# Autodesk Inventor assembly: test
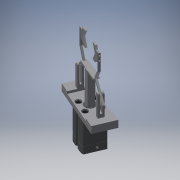
[picture p0: Inventor's stored thumbnail of the model, 180x180]
Saved by Autodesk Inventor 2017 (Build 210142000, 142)
## iProperties
Created: 2018-05-29
Part Number: test
Document SubType Name: Assembly
Designer: Pies
Author: Pies
## Documents named in this file (8)
- C:\Users\Pies\Desktop\Rzeczy\AGH\Semestr 2\ZIPK\Chwytak\Moj_Chwd_Pytak\Inventorowe chwytaki\test.iam
- C:\Users\Pies\Desktop\Rzeczy\AGH\Semestr 2\ZIPK\Chwytak\Moj_Chwd_Pytak\Inventorowe chwytaki\Ciągaczka.ipt
- C:\Users\Pies\Desktop\Rzeczy\AGH\Semestr 2\ZIPK\Chwytak\Moj_Chwd_Pytak\Inventorowe chwytaki\PIN.ipt
- C:\Users\Pies\Desktop\Rzeczy\AGH\Semestr 2\ZIPK\Chwytak\Moj_Chwd_Pytak\Inventorowe chwytaki\Ramię z łapką.iam
- C:\Users\Pies\Desktop\Rzeczy\AGH\Semestr 2\ZIPK\Chwytak\Moj_Chwd_Pytak\Inventorowe chwytaki\Podstawka.ipt
- C:\Users\Pies\Desktop\Rzeczy\AGH\Semestr 2\ZIPK\Chwytak\Moj_Chwd_Pytak\Inventorowe chwytaki\MOJ KOLNIERZ.ipt
- C:\Users\Pies\Desktop\Rzeczy\AGH\Semestr 2\ZIPK\Chwytak\Moj_Chwd_Pytak\Inventorowe chwytaki\Silownik\536236 ADN-20-15-A-P-A---(asm_0).iam
- C:\Users\Pies\Desktop\Rzeczy\AGH\Semestr 2\ZIPK\Chwytak\Moj_Chwd_Pytak\Inventorowe chwytaki\Kołnierz\DIN-6912 - M5x20(F).ipt
## Components (15 placed, 7 different names)
1. PIN:1 — Rigid:2
2. PIN:2 — Rigid:3
3. PIN:3 — Rigid:4
4. Ramię z łapką:1 [sub-assembly] — Rotational:1, Mate:13
5. Ramię z łapką:2 [sub-assembly] — Rotational:2, Mate:15
6. Ciągaczka:1 — Rotational:1, Rigid:2, Rotational:2, Rigid:3, Mate:10
7. Podstawka:1 — Mate:6, Mate:12, Mate:13, Rigid:5
8. Podstawka:2 — Mate:9, Mate:14, Mate:15, Rigid:4
9. MOJ KOLNIERZ:1 — Mate:6, Mate:9, Mate:10, Mate:12, Mate:14, Mate:19, Mate:20, Mate:23, Mate:24, Mate:25, Mate:26, Mate:28
10. PIN:4 — Rigid:5
11. 536236 ADN-20-15-A-P-A---(asm_0):1 [sub-assembly] — Mate:26, Mate:27, Mate:28
12. DIN-6912 - M5x20(F):1 — Mate:19
13. DIN-6912 - M5x20(F):2 — Mate:20
14. DIN-6912 - M5x20(F):3 — Mate:25, Mate:27
15. DIN-6912 - M5x20(F):4 — Mate:23, Mate:24
## Relationships (21: Mate 15, WeldJoint 4, RevoluteJoint 2)
- Rotational:1 [RevoluteJoint]: Ramię z łapką:1 ↔ Ciągaczka:1
- Rigid:2 [WeldJoint]: PIN:1 ↔ Ciągaczka:1
- Rotational:2 [RevoluteJoint]: Ramię z łapką:2 ↔ Ciągaczka:1
- Rigid:3 [WeldJoint]: PIN:2 ↔ Ciągaczka:1
- Mate:6: Podstawka:1 ↔ MOJ KOLNIERZ:1
- Mate:9: Podstawka:2 ↔ MOJ KOLNIERZ:1
- Mate:10: Ciągaczka:1 ↔ MOJ KOLNIERZ:1
- Mate:12: Podstawka:1 ↔ MOJ KOLNIERZ:1
- Mate:13: Ramię z łapką:1 ↔ Podstawka:1
- Mate:14: Podstawka:2 ↔ MOJ KOLNIERZ:1
- Mate:15: Ramię z łapką:2 ↔ Podstawka:2
- Rigid:4 [WeldJoint]: PIN:3 ↔ Podstawka:2
- Rigid:5 [WeldJoint]: Podstawka:1 ↔ PIN:4
- Mate:19: MOJ KOLNIERZ:1 ↔ DIN-6912 - M5x20(F):1
- Mate:20: MOJ KOLNIERZ:1 ↔ DIN-6912 - M5x20(F):2
- Mate:23: MOJ KOLNIERZ:1 ↔ DIN-6912 - M5x20(F):4
- Mate:24: MOJ KOLNIERZ:1 ↔ DIN-6912 - M5x20(F):4
- Mate:25: MOJ KOLNIERZ:1 ↔ DIN-6912 - M5x20(F):3
- Mate:26: MOJ KOLNIERZ:1 ↔ 536236 ADN-20-15-A-P-A---(asm_0):1
- Mate:27: 536236 ADN-20-15-A-P-A---(asm_0):1 ↔ DIN-6912 - M5x20(F):3
- Mate:28: MOJ KOLNIERZ:1 ↔ 536236 ADN-20-15-A-P-A---(asm_0):1
